# Autodesk Inventor assembly: 剪刀式升降
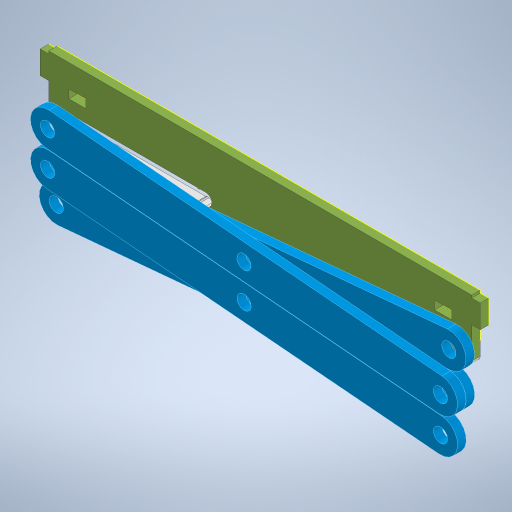
[picture p0: Inventor's stored thumbnail of the model, 512x512]
Saved by Autodesk Inventor 2023 (Build 270158000, 158)
## iProperties
Created: 2023-03-17
Part Number: 剪刀式升降
Document SubType Name: Assembly
Designer: may9c
Author: may9c
## Documents named in this file (3)
- D:\Areo_Rider_Cabin\Expansion\scisor lift.iam
- D:\Areo_Rider_Cabin\Expansion\link.ipt
- D:\Areo_Rider_Cabin\Expansion\chassis_1_2_1.ipt
## Components (5 placed, 2 different names)
1. link:1 — 插入:1, 插入:2, 插入:4
2. chassis_1_2_1:1 — 貼合:1, 貼合:2, 插入:1, 相切:1
3. link:2 — 插入:2, 插入:3, 相切:1
4. link:3 — 插入:3, 插入:5
5. link:4 — 插入:4, 插入:5
## Relationships (8: Insert 5, Mate 2, Tangent 1)
- 貼合:1 [Mate]: chassis_1_2_1:1
- 貼合:2 [Mate]: chassis_1_2_1:1
- 插入:1 [Insert]: link:1 ↔ chassis_1_2_1:1
- 插入:2 [Insert]: link:1 ↔ link:2
- 插入:3 [Insert]: link:2 ↔ link:3
- 插入:4 [Insert]: link:1 ↔ link:4
- 插入:5 [Insert]: link:3 ↔ link:4
- 相切:1 [Tangent]: chassis_1_2_1:1 ↔ link:2
